# Autodesk Inventor assembly: Cover_strip_fit_check
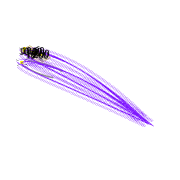
[picture p0: Inventor's stored thumbnail of the model, 180x180]
Saved by Autodesk Inventor 2022 (Build 260153000, 153)
## iProperties
Created: 2022-08-14
Part Number: Cover_strip_fit_check
Document SubType Name: Assembly
Designer: dell
Author: dell
## Documents named in this file (3)
- D:\xxxx\Uni\Part IV\MECHENG_700\Part_IV_project_CAD\Bird_skeleton_prototypes\Wing_drone_V1\Bird_wing_V2\Wing_cover\Cover_strip_fit_check.iam
- D:\xxxx\Uni\Part IV\MECHENG_700\Part_IV_project_CAD\Bird_skeleton_prototypes\Wing_drone_V1\Bird_wing_V2\Wing_cover\Radius_soft_cover.ipt
- D:\xxxx\Uni\Part IV\MECHENG_700\Part_IV_project_CAD\Bird_skeleton_prototypes\Wing_drone_V1\Bird_wing_V2\Wing_cover\Radius_cover_strip.ipt
## Components (2 placed, 2 different names)
1. Radius_soft_cover:1 — Flush:1
2. Radius_cover_strip:1 — Flush:1
## Relationships (1: Flush 1)
- Flush:1: Radius_soft_cover:1 ↔ Radius_cover_strip:1
